# Autodesk Inventor assembly: daVinciHead_OuterFrame
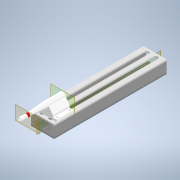
[picture p0: Inventor's stored thumbnail of the model, 180x180]
Saved by Autodesk Inventor 2022 (Build 260153000, 153)
## iProperties
Created: 2022-08-02
Part Number: daVinciHead_OuterFrame
Document SubType Name: Assembly
Designer: alexw
Author: alexw
## Documents named in this file (5)
- C:\Users\alexw\Documents\Inventor\Projects\03_CurrentProjects\MasterThesis\PSM_V1_Rillenkugellager\daVinciHead_OuterFrame.iam
- C:\Users\alexw\Documents\Inventor\Projects\03_CurrentProjects\MasterThesis\PSM_V1_Rillenkugellager\Slot profile.ipt
- C:\Users\alexw\Documents\Inventor\Projects\03_CurrentProjects\MasterThesis\PSM_V1_Rillenkugellager\Back plate profile.ipt
- C:\Users\alexw\Documents\Inventor\Projects\03_CurrentProjects\MasterThesis\PSM_V1_Rillenkugellager\Guide.ipt
- C:\Users\alexw\Documents\Inventor\Projects\03_CurrentProjects\MasterThesis\PSM_V1_Rillenkugellager\Ueberarbeiteter DaVincikopf\Fuehrungsschiene.ipt
## Components (4 placed, 4 different names)
1. Slot profile:1 — Fluchtend:6, Fluchtend:7, Passend:13
2. Back plate profile:1 — Fluchtend:1, Fluchtend:2, Fluchtend:4, Passend:12, Fluchtend:5
3. Guide:1 — Fluchtend:3
4. Fuehrungsschiene:1 — Fluchtend:4, Passend:12, Fluchtend:5, Fluchtend:6, Fluchtend:7, Passend:13
## Relationships (11: Flush 7, Mate 4)
- [Mate]: Slot profile:1 ↔ Guide:1
- [Mate]: Slot profile:1 ↔ Guide:1
- Fluchtend:1 [Flush]: Back plate profile:1
- Fluchtend:2 [Flush]: Back plate profile:1
- Fluchtend:3 [Flush]: Guide:1
- Fluchtend:4 [Flush]: Back plate profile:1 ↔ Fuehrungsschiene:1
- Passend:12 [Mate]: Back plate profile:1 ↔ Fuehrungsschiene:1
- Fluchtend:5 [Flush]: Back plate profile:1 ↔ Fuehrungsschiene:1
- Fluchtend:6 [Flush]: Slot profile:1 ↔ Fuehrungsschiene:1
- Fluchtend:7 [Flush]: Slot profile:1 ↔ Fuehrungsschiene:1
- Passend:13 [Mate]: Slot profile:1 ↔ Fuehrungsschiene:1
